# Autodesk Inventor assembly: ramp
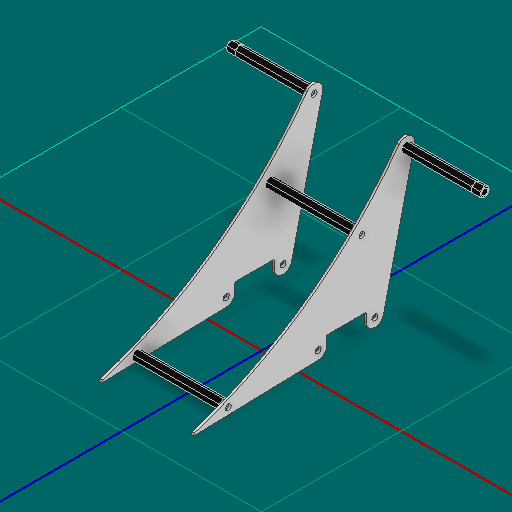
[picture p0: Inventor's stored thumbnail of the model, 512x512]
Saved by Autodesk Inventor 2025 (Build 290162000, 162)
## iProperties
Created: 2024-10-15
Part Number: ramp
Document SubType Name: Assembly
Designer: averey
Author: averey
## Documents named in this file (6)
- C:\Users\avere\vex_robotics_high_stakes\hardware\cad\bots\high_stakes_v2\intake\ramp.iam
- C:\Users\avere\vex_robotics_high_stakes\hardware\cad\bots\high_stakes_v2\intake\custom_parts\ramp.ipt
- C:\Users\avere\vex_robotics_high_stakes\hardware\cad\robpros_cad_lib\Structure\Standoff\Standoff .25.ipt
- C:\Users\avere\vex_robotics_high_stakes\hardware\cad\robpros_cad_lib\Structure\Standoff.ipt
- C:\Users\avere\vex_robotics_high_stakes\hardware\cad\robpros_cad_lib\Structure\Standoff\Standoff 2.00.ipt
- C:\Users\avere\vex_robotics_high_stakes\hardware\cad\robpros_cad_lib\Structure\Standoff\Standoff 2.50.ipt
## Components (8 placed, 4 different names)
1. ramp:1
2. ramp:2
3. Standoff .25:1
4. Standoff 2.00:2
5. Standoff .25:3
6. Standoff 2.00:4
7. Standoff 2.50:5
8. Standoff 2.50:6
## Relationships (5: Insert 5)
- [Insert]: Standoff .25:1 ↔ Standoff 2.00:2
- [Insert]: ramp:1 ↔ Standoff 2.00:2
- [Insert]: Standoff .25:3 ↔ Standoff 2.00:4
- [Insert]: ramp:2 ↔ Standoff 2.50:5
- [Insert]: ramp:2 ↔ Standoff 2.50:6
## Named parameters: d145_d143 = 0 mm
